# Autodesk Inventor assembly: optic_rail
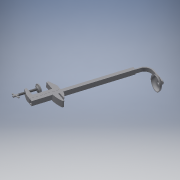
[picture p0: Inventor's stored thumbnail of the model, 180x180]
Saved by Autodesk Inventor 2019.3 (Build 233278000, 278)
## iProperties
Created: 2019-04-14
Part Number: optic_rail
Document SubType Name: Assembly
Designer: peter
Author: peter
## Documents named in this file (8)
- C:\Users\peter\OneDrive\Documents\Inventor\Automated Bar\optic_rail.iam
- C:\Users\peter\OneDrive\Documents\Inventor\Automated Bar\clamp.ipt
- C:\Users\peter\OneDrive\Documents\Inventor\Automated Bar\topbar.ipt
- C:\Users\peter\OneDrive\Documents\Inventor\Automated Bar\mainbar.ipt
- C:\Users\peter\OneDrive\Documents\Inventor\Automated Bar\cup.ipt
- C:\Users\peter\OneDrive\Documents\Inventor\Automated Bar\opticmount.ipt
- C:\Users\peter\OneDrive\Documents\Inventor\Automated Bar\clamp_cup.ipt
- C:\Users\peter\OneDrive\Documents\Inventor\Automated Bar\screw.ipt
## Components (7 placed, 7 different names)
1. clamp:1 — Mate:6, Mate:7, Mate:8, Mate:10, Mate:13, Mate:15
2. topbar:1 — Mate:11, Mate:12, Mate:16, Mate:17
3. mainbar:1 — Mate:6, Mate:7, Mate:8, Mate:9, Flush:1, Mate:16, Mate:17
4. cup:1 — Mate:11, Mate:12
5. opticmount:1 — Mate:9, Mate:10, Flush:1
6. clamp_cup:1 — Flush:2, Mate:14, Mate:15
7. screw:1 — Mate:13, Flush:2, Mate:14
## Relationships (14: Mate 12, Flush 2)
- Mate:6: clamp:1 ↔ mainbar:1
- Mate:7: clamp:1 ↔ mainbar:1
- Mate:8: clamp:1 ↔ mainbar:1
- Mate:9: mainbar:1 ↔ opticmount:1
- Mate:10: clamp:1 ↔ opticmount:1
- Flush:1 (-2 mm): mainbar:1 ↔ opticmount:1
- Mate:11: topbar:1 ↔ cup:1
- Mate:12: topbar:1 ↔ cup:1
- Mate:13: clamp:1 ↔ screw:1
- Flush:2: clamp_cup:1 ↔ screw:1
- Mate:14: clamp_cup:1 ↔ screw:1
- Mate:15 (22 mm): clamp:1 ↔ clamp_cup:1
- Mate:16 (0.5 mm): topbar:1 ↔ mainbar:1
- Mate:17: topbar:1 ↔ mainbar:1
